# Autodesk Inventor assembly: SUPPORT
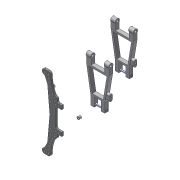
[picture p0: Inventor's stored thumbnail of the model, 180x180]
Saved by Autodesk Inventor 2016 (Build 200138000, 138)
## iProperties
Created: 2015-04-18
Part Number: SUPPORT
Document SubType Name: Assembly
Designer: Station9
Author: Station9
## Documents named in this file (5)
- E:\worldskills Project\Project Archive\AD\AD-6(94.01.29)WSC2011\SUPPORT.iam
- E:\worldskills Project\Project Archive\AD\AD-6(94.01.29)WSC2011\500-006.ipt
- E:\worldskills Project\Project Archive\AD\AD-6(94.01.29)WSC2011\307-320.ipt
- E:\worldskills Project\Project Archive\AD\AD-6(94.01.29)WSC2011\500-111.ipt
- E:\worldskills Project\Project Archive\AD\AD-6(94.01.29)WSC2011\500-120.ipt
## Components (7 placed, 4 different names)
1. 500-006:1 — Mate:1, Flush:1
2. 307-320:1 — Mate:1, Flush:1
3. 500-111:1
4. 500-120:1
5. 500-006:2 — Mate:2
6. 307-320:2 — Mate:2
7. 500-111:2
## Relationships (3: Mate 2, Flush 1)
- Mate:1: 500-006:1 ↔ 307-320:1
- Flush:1: 500-006:1 ↔ 307-320:1
- Mate:2: 500-006:2 ↔ 307-320:2
